# Autodesk Inventor assembly: motor_wheel_2
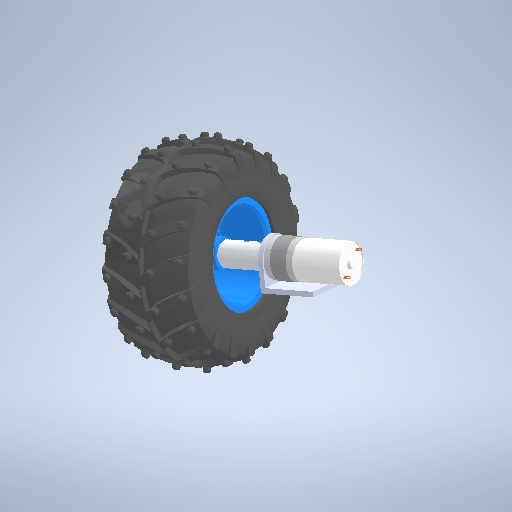
[picture p0: Inventor's stored thumbnail of the model, 512x512]
Saved by Autodesk Inventor 2025.3 (Build 293356030, 356C)
## iProperties
Created: 2026-06-28
Part Number: motor_wheel_2
Document SubType Name: Assembly
Designer: user
Author: user
## Documents named in this file (5)
- C:\Docs\shcool\dojo\Design_3\motor_wheel\motor_wheel_2.iam
- C:\Docs\shcool\dojo\Design_3\motor_wheel\Geared_motor.ipt
- C:\Docs\shcool\dojo\Design_3\motor_wheel\Hub-12-Eixo6_aluminio.ipt
- C:\Docs\shcool\dojo\Design_3\motor_wheel\motor bracket.ipt
- C:\Docs\shcool\dojo\Design_3\motor_wheel\Spiked Rubber Wheel 120mm.ipt
## Components (4 placed, 4 different names)
1. Geared_motor:1 — Insert:1
2. Hub-12-Eixo6_aluminio:1 — Mate:2, Mate:3, Mate:4, Mate:5
3. motor bracket:1 — Mate:2, Mate:3, Insert:1
4. Spiked Rubber Wheel 120mm:1 — Mate:4, Mate:5
## Relationships (5: Mate 4, Insert 1)
- Mate:2: Hub-12-Eixo6_aluminio:1 ↔ motor bracket:1
- Mate:3: Hub-12-Eixo6_aluminio:1 ↔ motor bracket:1
- Mate:4: Hub-12-Eixo6_aluminio:1 ↔ Spiked Rubber Wheel 120mm:1
- Mate:5: Hub-12-Eixo6_aluminio:1 ↔ Spiked Rubber Wheel 120mm:1
- Insert:1: Geared_motor:1 ↔ motor bracket:1
